# Autodesk Inventor assembly: main_assembly
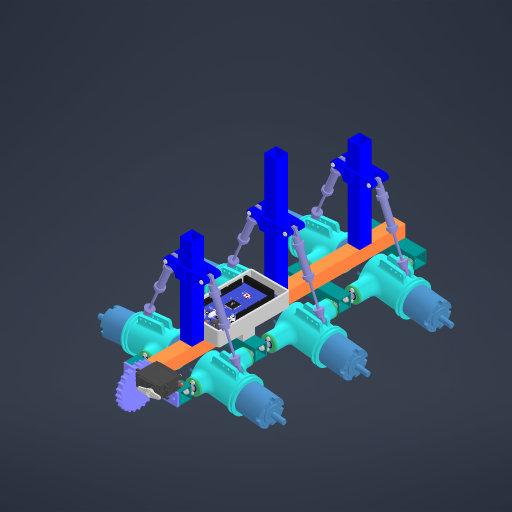
[picture p0: Inventor's stored thumbnail of the model, 512x512]
Saved by Autodesk Inventor 2024 (Build 280153000, 153)
## iProperties
Created: 2023-04-13
Part Number: main_assembly
Document SubType Name: Assembly
Designer: user
Author: user
## Documents named in this file (5)
- D:\Docs\Robot\3d\main_assembly.iam
- D:\Docs\Robot\3d\base\base_assembly.iam
- D:\Docs\Robot\3d\electronics\Arduino MEGA 2560 R3.ipt
- D:\Docs\Robot\3d\machine_body\front_box.ipt
- D:\Docs\Robot\3d\machine_body\manipulator_asembly.iam
## Components (4 placed, 4 different names)
1. base_assembly:1 [sub-assembly] — Совмещение:1, Совмещение:2, Совмещение:3, Совмещение:4, Заподлицо:1
2. Arduino MEGA 2560 R3:1
3. front_box:1 — Заподлицо:1
4. manipulator_asembly:1 [sub-assembly]
## Relationships (5: Mate 4, Flush 1)
- Совмещение:1 [Mate]: base_assembly:1
- Совмещение:2 [Mate]: base_assembly:1
- Совмещение:3 [Mate]: base_assembly:1
- Совмещение:4 [Mate]: base_assembly:1
- Заподлицо:1 [Flush]: base_assembly:1 ↔ front_box:1
